# Autodesk Inventor assembly: Robot_assembly_full
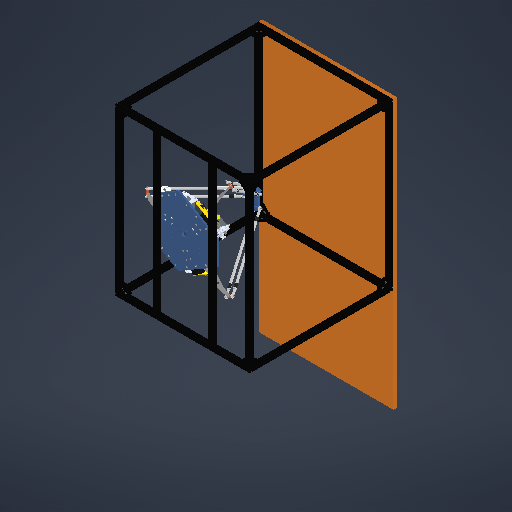
[picture p0: Inventor's stored thumbnail of the model, 512x512]
Saved by Autodesk Inventor 2027.1 (Build 311270010, 270A)
## iProperties
Created: 2026-08-09
Part Number: Robot_assembly_full
Document SubType Name: Assembly
Designer: MSI
Author: MSI
## Documents named in this file (35)
- C:\Users\MSI\Documents\MECHATRONICS\Tot_nghiep\Do_an_Delta.Robot_Dang_Rui_Bi\Thiết kế\Delta Part\Robot_assembly_full.iam
- C:\Users\MSI\Documents\MECHATRONICS\Tot_nghiep\Do_an_Delta.Robot_Dang_Rui_Bi\Thiết kế\Delta Part\tấm gỗ.ipt
- C:\Users\MSI\Documents\MECHATRONICS\Tot_nghiep\Do_an_Delta.Robot_Dang_Rui_Bi\Thiết kế\Delta Part\nhôm định hình 20x20_600.ipt
- C:\Users\MSI\Documents\MECHATRONICS\Tot_nghiep\Do_an_Delta.Robot_Dang_Rui_Bi\Thiết kế\Delta Part\nhôm định hình 20x20_700.ipt
- C:\Users\MSI\Documents\MECHATRONICS\Tot_nghiep\Do_an_Delta.Robot_Dang_Rui_Bi\Thiết kế\Delta Part\ke góc.ipt
- C:\Users\MSI\Documents\Inventor\Content Center Files\R2027\en-US\ISO 7380-1\ISO 7380-1 - M5 x 8.ipt
- C:\Users\MSI\Documents\MECHATRONICS\Tot_nghiep\Do_an_Delta.Robot_Dang_Rui_Bi\Thiết kế\Delta Part\nhôm định hình 20x20_600_có lỗ.ipt
- C:\Users\MSI\Documents\MECHATRONICS\Tot_nghiep\Do_an_Delta.Robot_Dang_Rui_Bi\Thiết kế\Delta Part\nhôm định hình 20x20_700_co lỗ1.ipt
- C:\Users\MSI\Documents\MECHATRONICS\Tot_nghiep\Do_an_Delta.Robot_Dang_Rui_Bi\Thiết kế\Delta Part\nhôm định hình 20x20_700_co lỗ2.ipt
- C:\Users\MSI\Documents\MECHATRONICS\Tot_nghiep\Do_an_Delta.Robot_Dang_Rui_Bi\Thiết kế\Delta Part\đế trên.ipt
- C:\Users\MSI\Documents\MECHATRONICS\Tot_nghiep\Do_an_Delta.Robot_Dang_Rui_Bi\Thiết kế\Delta Part\nhôm định hình đôi_gá link1.ipt
- C:\Users\MSI\Documents\MECHATRONICS\Tot_nghiep\Do_an_Delta.Robot_Dang_Rui_Bi\Thiết kế\Delta Part\Hộp trượt vòng bi.ipt
- C:\Users\MSI\Documents\MECHATRONICS\Tot_nghiep\Do_an_Delta.Robot_Dang_Rui_Bi\Thiết kế\Delta Part\trục đai.ipt
- C:\Users\MSI\Documents\MECHATRONICS\Tot_nghiep\Do_an_Delta.Robot_Dang_Rui_Bi\Thiết kế\Delta Part\mặt bích.ipt
- C:\Users\MSI\Documents\MECHATRONICS\Tot_nghiep\Do_an_Delta.Robot_Dang_Rui_Bi\Thiết kế\Delta Part\Link1.ipt
- C:\Users\MSI\Documents\MECHATRONICS\Tot_nghiep\Do_an_Delta.Robot_Dang_Rui_Bi\Thiết kế\Delta Part\khóa trục.ipt
- C:\Users\MSI\Documents\MECHATRONICS\Tot_nghiep\Do_an_Delta.Robot_Dang_Rui_Bi\Thiết kế\Delta Part\chốt khớp nối.ipt
- C:\Users\MSI\Documents\MECHATRONICS\Tot_nghiep\Do_an_Delta.Robot_Dang_Rui_Bi\Thiết kế\Delta Part\Base_E_buffer.ipt
- C:\Users\MSI\Documents\MECHATRONICS\Tot_nghiep\Do_an_Delta.Robot_Dang_Rui_Bi\Thiết kế\Delta Part\linh2_mawts traau.iam
- C:\Users\MSI\Documents\MECHATRONICS\Tot_nghiep\Do_an_Delta.Robot_Dang_Rui_Bi\Thiết kế\Delta Part\đế gá step.ipt
- C:\Users\MSI\Documents\MECHATRONICS\Tot_nghiep\Do_an_Delta.Robot_Dang_Rui_Bi\Thiết kế\Delta Part\nema23_57HS56\nema23.iam
- C:\Users\MSI\Documents\MECHATRONICS\Tot_nghiep\Do_an_Delta.Robot_Dang_Rui_Bi\Thiết kế\Delta Part\GT2_20T.ipt
- C:\Users\MSI\Documents\MECHATRONICS\Tot_nghiep\Do_an_Delta.Robot_Dang_Rui_Bi\Thiết kế\Delta Part\GT2_60.ipt
- C:\Users\MSI\Documents\Inventor\Content Center Files\R2027\en-US\AS 1427(05)\AS 1427 - M4 x 8(5) II.ipt
- C:\Users\MSI\Documents\Inventor\Content Center Files\R2027\en-US\AS 1427(05)\AS 1427 - M2.5 x 4(5) II.ipt
- C:\Users\MSI\Documents\Inventor\Content Center Files\R2027\en-US\AS 1427(05)\AS 1427 - M3.5 x 5(5) II.ipt
- C:\Users\MSI\Documents\Inventor\Content Center Files\R2027\en-US\AS 1427(05)\AS 1427 - M3 x 5(5) II.ipt
- C:\Users\MSI\Documents\Inventor\Content Center Files\R2027\en-US\AS 1427(05)\AS 1427 - M3 x 16(5) II.ipt
- C:\Users\MSI\Documents\Inventor\Content Center Files\R2027\en-US\AS 1427(05)\AS 1427 - M4 x 6(5) II.ipt
- C:\Users\MSI\Documents\Inventor\Content Center Files\R2027\en-US\ANSI B18.3.4M(1)\ANSI B18.3.4M - M3 x 0.5 x 45(2).ipt
- C:\Users\MSI\Documents\Inventor\Content Center Files\R2027\en-US\ANSI B18.2.4.2M\ANSI B18.2.4.2M - M3.5x0.6 - 6.ipt
- C:\Users\MSI\Documents\MECHATRONICS\Tot_nghiep\Do_an_Delta.Robot_Dang_Rui_Bi\Thiết kế\Tool_STL\Part1.ipt
- C:\Users\MSI\Documents\Inventor\Content Center Files\R2027\en-US\AS 1427(05)\AS 1427 - M4 x 10(5) II.ipt
- C:\Users\MSI\Documents\MECHATRONICS\Tot_nghiep\Do_an_Delta.Robot_Dang_Rui_Bi\Thiết kế\Delta Part\công tắc hành trình.ipt
- C:\Users\MSI\Documents\Inventor\Content Center Files\R2027\en-US\AS 1427(05)\AS 1427 - M4 x 16(5) II.ipt
## Components (233 placed, 34 different names)
1. tấm gỗ:1 — Flush:1, Mate:1, Flush:2, Mate:3, Flush:4, Mate:5, Flush:5, Flush:46, Flush:47, Flush:48
2. nhôm định hình 20x20_600:1 — Flush:1, Mate:1, Mate:2, Flush:3, Mate:4, Mate:10, Flush:10, Flush:11, Mate:11, Flush:12, Flush:13, Mate:21, Mate:22, Flush:24, Mate:27, Mate:30, Flush:28, Flush:47
3. nhôm định hình 20x20_700:1 — Mate:2, Flush:2, Flush:3, Mate:7, Mate:19, Mate:20, Flush:22, Flush:23, Mate:32, Flush:29, Mate:36, Flush:46
4. nhôm định hình 20x20_700:2 — Mate:3, Flush:4, Mate:4, Mate:6, Mate:8, Flush:6, Mate:23, Mate:25, Mate:28, Mate:38, Flush:48
5. nhôm định hình 20x20_600:2 — Mate:5, Mate:6, Mate:7, Flush:5, Flush:7, Mate:9, Flush:8, Flush:9, Mate:18, Mate:24, Flush:25, Mate:35, Mate:40
6. nhôm định hình 20x20_600:3 — Mate:10, Flush:10, Flush:11, Mate:31, Mate:33, Mate:54, Mate:56, Flush:41, Flush:50, Flush:53, Flush:54
7. nhôm định hình 20x20_600:4 — Mate:11, Flush:12, Flush:13, Mate:26, Flush:26, Mate:29, Flush:27, Mate:50, Mate:52, Flush:55, Flush:57, Flush:73
8. nhôm định hình 20x20_600:5 — Mate:9, Flush:8, Flush:9, Mate:34, Flush:30, Mate:37, Flush:31, Mate:43, Flush:34, Mate:44, Mate:67, Flush:59
9. nhôm định hình 20x20_600:6 — Mate:8, Flush:6, Flush:7, Mate:39, Flush:32, Mate:41, Flush:33, Mate:46, Flush:36, Mate:48, Flush:58
10. nhôm định hình 20x20_700:3 — Mate:45, Flush:35, Mate:57, Mate:58, Mate:60, Flush:49, Flush:60, Flush:67, Mate:73
11. nhôm định hình 20x20_700:4 — Mate:49, Flush:37, Mate:51, Flush:38, Mate:63, Flush:44, Mate:65, Mate:66, Flush:56, Flush:61, Flush:68, Flush:70
12. ke góc:1 — Mate:28, Mate:29, Flush:27, Insert:23, Insert:24
13. ke góc:2 — Mate:32, Mate:33, Flush:29, Insert:31, Insert:32
14. ke góc:3 — Mate:38, Mate:39, Flush:32, Insert:5, Insert:6, Insert:9
15. ke góc:4 — Mate:36, Mate:37, Flush:31, Insert:12, Insert:13
16. ke góc:5 — Mate:34, Mate:35, Flush:30, Insert:16, Insert:17
17. ke góc:6 — Mate:26, Mate:27, Flush:26, Insert:21, Insert:22
18. ke góc:7 — Mate:24, Mate:25, Flush:25, Insert:1, Insert:2, Insert:3, Insert:4
19. ke góc:8 — Mate:18, Mate:19, Flush:23, Insert:14, Insert:15
20. ke góc:9 — Mate:22, Flush:24, Mate:23, Insert:25, Insert:26
21. ke góc:10 — Mate:20, Mate:21, Flush:22, Insert:29, Insert:30
22. ke góc:11 — Mate:30, Mate:31, Flush:28, Insert:33, Insert:34
23. ke góc:12 — Mate:46, Flush:36, Insert:39, Insert:40, Flush:63, Mate:74
24. ke góc:13 — Mate:58, Insert:54, Insert:55, Flush:65, Mate:72
25. ke góc:14 — Mate:56, Mate:57, Flush:41, Insert:47, Insert:52
26. ke góc:15 — Mate:52, Insert:41, Insert:42, Flush:73, Mate:70
27. ke góc:16 — Mate:48, Mate:49, Flush:37, Insert:35, Insert:37
28. ke góc:17 — Mate:50, Mate:51, Flush:38, Insert:45, Insert:46
29. ke góc:18 — Mate:44, Mate:45, Flush:35, Insert:57, Insert:58
30. ke góc:19 — Mate:43, Flush:34, Insert:53, Insert:56, Flush:62, Mate:75
31. ke góc:20 — Mate:54, Insert:50, Insert:51, Mate:69, Flush:72
32. ke góc:21 — Mate:40, Mate:41, Flush:33, Insert:7, Insert:8
33. ke góc:22 — Mate:60, Insert:48, Insert:49, Flush:66, Flush:67, Mate:76
34. ke góc:23 — Mate:63, Flush:44, Insert:43, Insert:44, Mate:68, Flush:68, Flush:69
35. ke góc:24 — Mate:65, Insert:36, Insert:38, Flush:64, Flush:70, Flush:71, Mate:71
36. ISO 7380-1 M5 x 8:1 — Insert:1
37. ISO 7380-1 M5 x 8:2 — Insert:2
38. ISO 7380-1 M5 x 8:3 — Insert:3
39. ISO 7380-1 M5 x 8:4 — Insert:4
40. ISO 7380-1 M5 x 8:5 — Insert:5
41. ISO 7380-1 M5 x 8:6 — Insert:6
42. ISO 7380-1 M5 x 8:7 — Insert:7
43. ISO 7380-1 M5 x 8:8 — Insert:8
44. ISO 7380-1 M5 x 8:9 — Insert:9
45. ISO 7380-1 M5 x 8:12 — Insert:12
46. ISO 7380-1 M5 x 8:13 — Insert:13
47. ISO 7380-1 M5 x 8:14 — Insert:14
48. ISO 7380-1 M5 x 8:15 — Insert:15
49. ISO 7380-1 M5 x 8:16 — Insert:16
50. ISO 7380-1 M5 x 8:17 — Insert:17
51. ISO 7380-1 M5 x 8:22 — Insert:21
52. ISO 7380-1 M5 x 8:23 — Insert:22
53. ISO 7380-1 M5 x 8:24 — Insert:23
54. ISO 7380-1 M5 x 8:25 — Insert:24
55. ISO 7380-1 M5 x 8:26 — Insert:25
56. ISO 7380-1 M5 x 8:27 — Insert:26
57. ISO 7380-1 M5 x 8:30 — Insert:29
58. ISO 7380-1 M5 x 8:31 — Insert:30
59. ISO 7380-1 M5 x 8:32 — Insert:31
60. ISO 7380-1 M5 x 8:33 — Insert:32
61. ISO 7380-1 M5 x 8:34 — Insert:33
62. ISO 7380-1 M5 x 8:35 — Insert:34
63. ISO 7380-1 M5 x 8:36 — Insert:35
64. ISO 7380-1 M5 x 8:37 — Insert:36
65. ISO 7380-1 M5 x 8:38 — Insert:37
66. ISO 7380-1 M5 x 8:39 — Insert:38
67. ISO 7380-1 M5 x 8:40 — Insert:39
68. ISO 7380-1 M5 x 8:41 — Insert:40
69. ISO 7380-1 M5 x 8:42 — Insert:41
70. ISO 7380-1 M5 x 8:43 — Insert:42
71. ISO 7380-1 M5 x 8:44 — Insert:43
72. ISO 7380-1 M5 x 8:45 — Insert:44
73. ISO 7380-1 M5 x 8:46 — Insert:45
74. ISO 7380-1 M5 x 8:47 — Insert:46
75. ISO 7380-1 M5 x 8:48 — Insert:47
76. ISO 7380-1 M5 x 8:49 — Insert:48
77. ISO 7380-1 M5 x 8:50 — Insert:49
78. ISO 7380-1 M5 x 8:51 — Insert:50
79. ISO 7380-1 M5 x 8:52 — Insert:51
80. ISO 7380-1 M5 x 8:53 — Insert:52
81. ISO 7380-1 M5 x 8:54 — Insert:53
82. ISO 7380-1 M5 x 8:55 — Insert:54
83. ISO 7380-1 M5 x 8:56 — Insert:55
84. ISO 7380-1 M5 x 8:57 — Insert:56
85. ISO 7380-1 M5 x 8:58 — Insert:57
86. ISO 7380-1 M5 x 8:59 — Insert:58
87. nhôm định hình 20x20_600_có lỗ:1 — Mate:66, Mate:67, Flush:49, Flush:58, Flush:59, Flush:60, Flush:61, Flush:62, Flush:63, Flush:64, Flush:65, Flush:71, Mate:71, Mate:72, Mate:73, Mate:74, Mate:75, Mate:78, Flush:74, Mate:79
88. nhôm định hình 20x20_600_có lỗ:2 — Mate:68, Mate:69, Flush:50, Flush:53, Flush:54, Flush:55, Flush:56, Flush:57, Flush:66, Flush:69, Flush:72, Mate:70, Mate:76, Mate:77, Flush:75, Mate:80
89. nhôm định hình 20x20_700_co lỗ1:1 — Mate:77, Mate:78, Flush:74, Mate:81
90. nhôm định hình 20x20_700_co lỗ2:1 — Mate:79, Flush:75, Mate:80, Flush:76, Mate:82, Insert:104, Insert:105, Insert:106
91. đế trên:1 — Mate:81, Flush:76, Mate:82, Mate:83, Mate:84, Mate:85, Mate:95, Mate:96, Mate:97, Mate:98, Mate:99, Mate:100, Insert:94, Insert:95, Insert:96, Insert:97, Insert:98, Insert:99, Insert:100, Insert:101, Insert:103, Insert:107, Insert:108, Insert:109, Insert:110, Insert:111, Insert:141, Insert:142, Insert:143, Insert:144, Insert:145, Insert:146, Insert:147, Insert:148, Insert:149, Insert:150, Insert:151, Insert:152, Insert:153
92. nhôm định hình đôi_gá link1:1 — Mate:83, Mate:84, Mate:85, Mate:86, Flush:77, Flush:82, Mate:236, Flush:83, Flush:84, Flush:103, Flush:104, Mate:265
93. Hộp trượt vòng bi:1 — Mate:86, Flush:77, Mate:88, Mate:89, Mate:122, Flush:82, Insert:90, Insert:91, Insert:92, Insert:93
94. trục đai:1 — Mate:88, Mate:89, Mate:90, Mate:121, Mate:209, Mate:256
95. mặt bích:1 — Mate:90, Mate:92, Mate:93, Mate:94, Mate:209
96. Link1:1 — Mate:92, Mate:93, Mate:94, Mate:129, Mate:130, Mate:131, Mate:132, Insert:79, Insert:80, Insert:81, Insert:82
97. nhôm định hình đôi_gá link1:2 — Mate:98, Mate:99, Mate:100, Mate:101, Flush:78, Flush:80, Flush:87, Mate:242, Flush:88, Mate:266, Flush:105, Flush:106
98. nhôm định hình đôi_gá link1:3 — Mate:95, Mate:96, Mate:97, Mate:103, Flush:79, Flush:81, Mate:239, Flush:86, Flush:94, Mate:267, Flush:107, Flush:108
99. Hộp trượt vòng bi:2 — Mate:101, Flush:78, Mate:107, Mate:124, Flush:80, Insert:83, Insert:84, Insert:85, Insert:86
100. Hộp trượt vòng bi:3 — Mate:103, Flush:79, Mate:105, Mate:106, Mate:120, Flush:81, Mate:261, Mate:262, Insert:87, Insert:88, Insert:89
101. trục đai:2 — Mate:105, Mate:106, Mate:111, Mate:119, Mate:208, Mate:257
102. trục đai:3 — Mate:107, Mate:109, Mate:123, Mate:255
103. mặt bích:2 — Mate:111, Mate:116, Mate:117, Mate:118, Mate:208
104. mặt bích:3 — Mate:109, Mate:113, Mate:114, Mate:115
105. Link1:2 — Mate:113, Mate:114, Mate:115, Mate:133, Mate:134, Mate:135, Mate:136, Insert:75, Insert:76, Insert:77, Insert:78
106. Link1:3 — Mate:116, Mate:117, Mate:118, Mate:125, Mate:126, Mate:127, Mate:128, Insert:71, Insert:72, Insert:73, Insert:74
107. khóa trục:1 — Mate:119, Mate:120, Mate:258
108. khóa trục:2 — Mate:121, Mate:122, Mate:259
109. khóa trục:3 — Mate:123, Mate:124, Mate:260
110. chốt khớp nối:1 — Mate:125, Mate:126, Mate:215
111. chốt khớp nối:2 — Mate:131, Mate:132, Mate:212, Mate:213
112. chốt khớp nối:3 — Mate:127, Mate:128, Mate:214, Mate:216, Mate:217
113. chốt khớp nối:4 — Mate:135, Mate:136, Mate:218, Mate:219
114. chốt khớp nối:5 — Mate:133, Mate:134, Mate:220, Mate:221
115. chốt khớp nối:6 — Mate:129, Mate:130, Mate:210, Mate:211
116. linh2_mawts traau:1 [sub-assembly] — Mate:210, Mate:211, Mate:232, Mate:233, Insert:131, Insert:132
117. linh2_mawts traau:2 [sub-assembly] — Mate:218, Mate:219, Mate:227, Mate:228, Insert:129, Insert:133
118. linh2_mawts traau:3 [sub-assembly] — Mate:216, Mate:217, Mate:224, Mate:231, Insert:126, Mate:263, Mate:264
119. linh2_mawts traau:4 [sub-assembly] — Mate:220, Mate:221, Mate:225, Mate:226, Mate:229, Insert:127, Insert:128
120. linh2_mawts traau:5 [sub-assembly] — Mate:214, Mate:215, Mate:222, Mate:223, Mate:230, Insert:130, Insert:134
121. linh2_mawts traau:6 [sub-assembly] — Mate:212, Mate:213, Mate:234, Mate:235, Insert:124, Insert:125
122. Base_E_buffer:1 — Mate:222, Mate:223, Mate:224, Mate:225, Mate:226, Mate:227, Mate:228, Mate:229, Mate:230, Mate:231, Mate:232, Mate:233, Mate:234, Mate:235
123. nema23:1 [sub-assembly] — Mate:237, Mate:251, Mate:252, Flush:97
124. đế gá step:1 — Mate:236, Flush:83, Flush:84, Mate:237, Mate:251, Insert:63, Insert:64, Insert:65, Insert:66
125. đế gá step:2 — Mate:239, Flush:86, Flush:94, Mate:249, Flush:96, Insert:59, Insert:60, Insert:61, Insert:62
126. đế gá step:3 — Flush:87, Mate:242, Flush:88, Mate:243, Flush:95, Insert:67, Insert:68, Insert:69, Insert:70
127. nema23:3 [sub-assembly] — Mate:243, Flush:95, Mate:254, Flush:99
128. nema23:4 [sub-assembly] — Mate:249, Flush:96, Mate:253, Flush:98
129. GT2_20T:1 — Mate:253, Flush:98, Flush:102
130. GT2_20T:2 — Mate:252, Flush:97, Flush:101
131. GT2_20T:3 — Mate:254, Flush:99, Flush:100
132. GT2_60:1 — Mate:257, Flush:102
133. GT2_60:2 — Mate:255, Flush:100
134. GT2_60:3 — Mate:256, Flush:101
135. AS 1427 H - Metric M4 x 8:1 — Insert:59
136. AS 1427 H - Metric M4 x 8:2 — Insert:60
137. AS 1427 H - Metric M4 x 8:3 — Insert:61
138. AS 1427 H - Metric M4 x 8:4 — Insert:62
139. AS 1427 H - Metric M4 x 8:5 — Insert:63
140. AS 1427 H - Metric M4 x 8:6 — Insert:64
141. AS 1427 H - Metric M4 x 8:7 — Insert:65
142. AS 1427 H - Metric M4 x 8:8 — Insert:66
143. AS 1427 H - Metric M4 x 8:9 — Insert:67
144. AS 1427 H - Metric M4 x 8:10 — Insert:68
145. AS 1427 H - Metric M4 x 8:11 — Insert:69
146. AS 1427 H - Metric M4 x 8:12 — Insert:70
147. AS 1427 H - Metric M2.5 x 4:1 — Insert:71
148. AS 1427 H - Metric M2.5 x 4:2 — Insert:72
149. AS 1427 H - Metric M2.5 x 4:3 — Insert:73
150. AS 1427 H - Metric M2.5 x 4:4 — Insert:74
151. AS 1427 H - Metric M2.5 x 4:5 — Insert:75
152. AS 1427 H - Metric M2.5 x 4:6 — Insert:76
153. AS 1427 H - Metric M2.5 x 4:7 — Insert:77
154. AS 1427 H - Metric M2.5 x 4:8 — Insert:78
155. AS 1427 H - Metric M2.5 x 4:9 — Insert:79
156. AS 1427 H - Metric M2.5 x 4:10 — Insert:80
157. AS 1427 H - Metric M2.5 x 4:11 — Insert:81
158. AS 1427 H - Metric M2.5 x 4:12 — Insert:82
159. AS 1427 H - Metric M3.5 x 5:1 — Mate:258
160. AS 1427 H - Metric M3.5 x 5:2 — Mate:259
161. AS 1427 H - Metric M3.5 x 5:3 — Mate:260
162. AS 1427 H - Metric M3 x 5:1 — Insert:83
163. AS 1427 H - Metric M3 x 5:2 — Insert:84
164. AS 1427 H - Metric M3 x 5:3 — Insert:85
165. AS 1427 H - Metric M3 x 5:4 — Insert:86
166. AS 1427 H - Metric M3 x 5:5 — Mate:261, Mate:262
167. AS 1427 H - Metric M3 x 5:6 — Insert:87
168. AS 1427 H - Metric M3 x 5:7 — Insert:88
169. AS 1427 H - Metric M3 x 16:1 — Insert:89
170. AS 1427 H - Metric M3 x 16:2 — Insert:90
171. AS 1427 H - Metric M3 x 16:3 — Insert:91
172. AS 1427 H - Metric M3 x 16:4 — Insert:92
173. AS 1427 H - Metric M3 x 16:5 — Insert:93
174. AS 1427 H - Metric M4 x 6:1 — Insert:94
175. AS 1427 H - Metric M4 x 6:2 — Insert:95
176. AS 1427 H - Metric M4 x 6:3 — Insert:96
177. AS 1427 H - Metric M4 x 6:4 — Insert:97
178. AS 1427 H - Metric M4 x 6:5 — Insert:98
179. AS 1427 H - Metric M4 x 6:6 — Insert:99
180. AS 1427 H - Metric M4 x 6:7 — Insert:100
181. AS 1427 H - Metric M4 x 6:8 — Insert:101
182. AS 1427 H - Metric M4 x 6:10 — Insert:103
183. AS 1427 H - Metric M4 x 6:11 — Insert:104
184. AS 1427 H - Metric M4 x 6:12 — Insert:105
185. AS 1427 H - Metric M4 x 6:13 — Insert:106
186. AS 1427 H - Metric M4 x 6:14 — Insert:107
187. AS 1427 H - Metric M4 x 6:15 — Insert:108
188. AS 1427 H - Metric M4 x 6:16 — Insert:109
189. AS 1427 H - Metric M4 x 6:17 — Insert:110
190. AS 1427 H - Metric M4 x 6:18 — Insert:111
191. Broached Hexagon Socket Button Head Cap Screw - Metric M3 x 0.5 x 45:1 — Insert:124
192. Broached Hexagon Socket Button Head Cap Screw - Metric M3 x 0.5 x 45:2 — Insert:125
193. Broached Hexagon Socket Button Head Cap Screw - Metric M3 x 0.5 x 45:3 — Insert:126
194. Broached Hexagon Socket Button Head Cap Screw - Metric M3 x 0.5 x 45:4 — Mate:263, Mate:264
195. Broached Hexagon Socket Button Head Cap Screw - Metric M3 x 0.5 x 45:5 — Insert:127
196. Broached Hexagon Socket Button Head Cap Screw - Metric M3 x 0.5 x 45:6 — Insert:128
197. ANSI B18.2.4.2M M3.5x0.6:1 — Insert:129
198. ANSI B18.2.4.2M M3.5x0.6:2 — Insert:130
199. ANSI B18.2.4.2M M3.5x0.6:3 — Insert:131
200. ANSI B18.2.4.2M M3.5x0.6:4 — Insert:132
201. ANSI B18.2.4.2M M3.5x0.6:5 — Insert:133
202. ANSI B18.2.4.2M M3.5x0.6:6 — Insert:134
203. Part1:1 — Mate:266, Flush:105, Flush:106, Insert:139, Insert:140, Mate:274, Mate:275, Mate:276
204. Part1:2 — Mate:267, Flush:107, Flush:108, Insert:135, Insert:136, Mate:271, Mate:272, Mate:273
205. Part1:3 — Flush:103, Flush:104, Mate:265, Insert:137, Insert:138, Mate:268, Mate:269, Mate:270
206. AS 1427 H - Metric M4 x 10:1 — Insert:135
207. AS 1427 H - Metric M4 x 10:2 — Insert:136
208. AS 1427 H - Metric M4 x 10:3 — Insert:137
209. AS 1427 H - Metric M4 x 10:4 — Insert:138
210. AS 1427 H - Metric M4 x 10:5 — Insert:139
211. AS 1427 H - Metric M4 x 10:6 — Insert:140
212. công tắc hành trình:1 — Mate:271, Mate:272, Mate:273, Insert:154, Insert:155
213. công tắc hành trình:2 — Mate:274, Mate:275, Mate:276, Insert:156, Insert:157
214. công tắc hành trình:3 — Mate:268, Mate:269, Mate:270, Insert:158, Insert:159
215. AS 1427 H - Metric M4 x 16:1 — Insert:141
216. AS 1427 H - Metric M4 x 16:2 — Insert:142
217. AS 1427 H - Metric M4 x 16:3 — Insert:143
218. AS 1427 H - Metric M4 x 16:4 — Insert:144
219. AS 1427 H - Metric M4 x 16:5 — Insert:145
220. AS 1427 H - Metric M4 x 16:6 — Insert:146
221. AS 1427 H - Metric M4 x 16:7 — Insert:147
222. AS 1427 H - Metric M4 x 16:8 — Insert:148
223. AS 1427 H - Metric M4 x 16:9 — Insert:149
224. AS 1427 H - Metric M4 x 16:10 — Insert:150
225. AS 1427 H - Metric M4 x 16:11 — Insert:151
226. AS 1427 H - Metric M4 x 10:7 — Insert:152
227. AS 1427 H - Metric M4 x 16:12 — Insert:153
228. AS 1427 H - Metric M3 x 5:8 — Insert:154
229. AS 1427 H - Metric M3 x 5:9 — Insert:155
230. AS 1427 H - Metric M3 x 5:10 — Insert:156
231. AS 1427 H - Metric M3 x 5:11 — Insert:157
232. AS 1427 H - Metric M3 x 5:12 — Insert:158
233. AS 1427 H - Metric M3 x 5:13 — Insert:159
## Relationships (401: Mate 175, Insert 139, Flush 87)
- Flush:1: tấm gỗ:1 ↔ nhôm định hình 20x20_600:1
- Mate:1: tấm gỗ:1 ↔ nhôm định hình 20x20_600:1
- Mate:2: nhôm định hình 20x20_600:1 ↔ nhôm định hình 20x20_700:1
- Flush:2: tấm gỗ:1 ↔ nhôm định hình 20x20_700:1
- Flush:3: nhôm định hình 20x20_600:1 ↔ nhôm định hình 20x20_700:1
- Mate:3: tấm gỗ:1 ↔ nhôm định hình 20x20_700:2
- Flush:4: tấm gỗ:1 ↔ nhôm định hình 20x20_700:2
- Mate:4: nhôm định hình 20x20_600:1 ↔ nhôm định hình 20x20_700:2
- Mate:5: tấm gỗ:1 ↔ nhôm định hình 20x20_600:2
- Mate:6: nhôm định hình 20x20_700:2 ↔ nhôm định hình 20x20_600:2
- Mate:7: nhôm định hình 20x20_700:1 ↔ nhôm định hình 20x20_600:2
- Flush:5: tấm gỗ:1 ↔ nhôm định hình 20x20_600:2
- Mate:8: nhôm định hình 20x20_700:2 ↔ nhôm định hình 20x20_600:6
- Flush:6: nhôm định hình 20x20_700:2 ↔ nhôm định hình 20x20_600:6
- Flush:7: nhôm định hình 20x20_600:2 ↔ nhôm định hình 20x20_600:6
- Mate:9: nhôm định hình 20x20_600:2 ↔ nhôm định hình 20x20_600:5
- Flush:8: nhôm định hình 20x20_600:2 ↔ nhôm định hình 20x20_600:5
- Flush:9: nhôm định hình 20x20_600:2 ↔ nhôm định hình 20x20_600:5
- Mate:10: nhôm định hình 20x20_600:1 ↔ nhôm định hình 20x20_600:3
- Flush:10: nhôm định hình 20x20_600:1 ↔ nhôm định hình 20x20_600:3
- Flush:11: nhôm định hình 20x20_600:1 ↔ nhôm định hình 20x20_600:3
- Mate:11: nhôm định hình 20x20_600:1 ↔ nhôm định hình 20x20_600:4
- Flush:12: nhôm định hình 20x20_600:1 ↔ nhôm định hình 20x20_600:4
- Flush:13: nhôm định hình 20x20_600:1 ↔ nhôm định hình 20x20_600:4
- Mate:18: nhôm định hình 20x20_600:2 ↔ ke góc:8
- Mate:19: nhôm định hình 20x20_700:1 ↔ ke góc:8
- Mate:20: nhôm định hình 20x20_700:1 ↔ ke góc:10
- Mate:21: nhôm định hình 20x20_600:1 ↔ ke góc:10
- Flush:22: nhôm định hình 20x20_700:1 ↔ ke góc:10
- Flush:23: nhôm định hình 20x20_700:1 ↔ ke góc:8
- Mate:22: nhôm định hình 20x20_600:1 ↔ ke góc:9
- Flush:24: nhôm định hình 20x20_600:1 ↔ ke góc:9
- Mate:23: nhôm định hình 20x20_700:2 ↔ ke góc:9
- Mate:24: nhôm định hình 20x20_600:2 ↔ ke góc:7
- Mate:25: nhôm định hình 20x20_700:2 ↔ ke góc:7
- Flush:25: nhôm định hình 20x20_600:2 ↔ ke góc:7
- Mate:26: nhôm định hình 20x20_600:4 ↔ ke góc:6
- Mate:27: nhôm định hình 20x20_600:1 ↔ ke góc:6
- Flush:26: nhôm định hình 20x20_600:4 ↔ ke góc:6
- Mate:28: nhôm định hình 20x20_700:2 ↔ ke góc:1
- Mate:29: nhôm định hình 20x20_600:4 ↔ ke góc:1
- Flush:27: nhôm định hình 20x20_600:4 ↔ ke góc:1
- Mate:30: nhôm định hình 20x20_600:1 ↔ ke góc:11
- Mate:31: nhôm định hình 20x20_600:3 ↔ ke góc:11
- Flush:28: nhôm định hình 20x20_600:1 ↔ ke góc:11
- Mate:32: nhôm định hình 20x20_700:1 ↔ ke góc:2
- Mate:33: nhôm định hình 20x20_600:3 ↔ ke góc:2
- Flush:29: nhôm định hình 20x20_700:1 ↔ ke góc:2
- Mate:34: nhôm định hình 20x20_600:5 ↔ ke góc:5
- Mate:35: nhôm định hình 20x20_600:2 ↔ ke góc:5
- Flush:30: nhôm định hình 20x20_600:5 ↔ ke góc:5
- Mate:36: nhôm định hình 20x20_700:1 ↔ ke góc:4
- Mate:37: nhôm định hình 20x20_600:5 ↔ ke góc:4
- Flush:31: nhôm định hình 20x20_600:5 ↔ ke góc:4
- Mate:38: nhôm định hình 20x20_700:2 ↔ ke góc:3
- Mate:39: nhôm định hình 20x20_600:6 ↔ ke góc:3
- Flush:32: nhôm định hình 20x20_600:6 ↔ ke góc:3
- Mate:40: nhôm định hình 20x20_600:2 ↔ ke góc:21
- Mate:41: nhôm định hình 20x20_600:6 ↔ ke góc:21
- Flush:33: nhôm định hình 20x20_600:6 ↔ ke góc:21
- Mate:43: nhôm định hình 20x20_600:5 ↔ ke góc:19
- Flush:34: nhôm định hình 20x20_600:5 ↔ ke góc:19
- Mate:44: nhôm định hình 20x20_600:5 ↔ ke góc:18
- Mate:45: nhôm định hình 20x20_700:3 ↔ ke góc:18
- Flush:35: nhôm định hình 20x20_700:3 ↔ ke góc:18
- Mate:46: nhôm định hình 20x20_600:6 ↔ ke góc:12
- Flush:36: nhôm định hình 20x20_600:6 ↔ ke góc:12
- Mate:48: nhôm định hình 20x20_600:6 ↔ ke góc:16
- Mate:49: nhôm định hình 20x20_700:4 ↔ ke góc:16
- Flush:37: nhôm định hình 20x20_700:4 ↔ ke góc:16
- Mate:50: nhôm định hình 20x20_600:4 ↔ ke góc:17
- Mate:51: nhôm định hình 20x20_700:4 ↔ ke góc:17
- Flush:38: nhôm định hình 20x20_700:4 ↔ ke góc:17
- Mate:52: nhôm định hình 20x20_600:4 ↔ ke góc:15
- Mate:54: nhôm định hình 20x20_600:3 ↔ ke góc:20
- Mate:56: nhôm định hình 20x20_600:3 ↔ ke góc:14
- Mate:57: nhôm định hình 20x20_700:3 ↔ ke góc:14
- Flush:41: nhôm định hình 20x20_600:3 ↔ ke góc:14
- Mate:58: nhôm định hình 20x20_700:3 ↔ ke góc:13
- Mate:60: nhôm định hình 20x20_700:3 ↔ ke góc:22
- Mate:63: nhôm định hình 20x20_700:4 ↔ ke góc:23
- Flush:44: nhôm định hình 20x20_700:4 ↔ ke góc:23
- Mate:65: nhôm định hình 20x20_700:4 ↔ ke góc:24
- Insert:1: ke góc:7 ↔ ISO 7380-1 M5 x 8:1
- Insert:2: ke góc:7 ↔ ISO 7380-1 M5 x 8:2
- Insert:3: ke góc:7 ↔ ISO 7380-1 M5 x 8:3
- Insert:4: ke góc:7 ↔ ISO 7380-1 M5 x 8:4
- Insert:5: ke góc:3 ↔ ISO 7380-1 M5 x 8:5
- Insert:6: ke góc:3 ↔ ISO 7380-1 M5 x 8:6
- Insert:7: ke góc:21 ↔ ISO 7380-1 M5 x 8:7
- Insert:8: ke góc:21 ↔ ISO 7380-1 M5 x 8:8
- Insert:9: ke góc:3 ↔ ISO 7380-1 M5 x 8:9
- Insert:12: ke góc:4 ↔ ISO 7380-1 M5 x 8:12
- Insert:13: ke góc:4 ↔ ISO 7380-1 M5 x 8:13
- Insert:14: ke góc:8 ↔ ISO 7380-1 M5 x 8:14
- Insert:15: ke góc:8 ↔ ISO 7380-1 M5 x 8:15
- Insert:16: ke góc:5 ↔ ISO 7380-1 M5 x 8:16
- Insert:17: ke góc:5 ↔ ISO 7380-1 M5 x 8:17
- Insert:21: ke góc:6 ↔ ISO 7380-1 M5 x 8:22
- Insert:22: ke góc:6 ↔ ISO 7380-1 M5 x 8:23
- Insert:23: ke góc:1 ↔ ISO 7380-1 M5 x 8:24
- Insert:24: ke góc:1 ↔ ISO 7380-1 M5 x 8:25
- Insert:25: ke góc:9 ↔ ISO 7380-1 M5 x 8:26
- Insert:26: ke góc:9 ↔ ISO 7380-1 M5 x 8:27
- Insert:29: ke góc:10 ↔ ISO 7380-1 M5 x 8:30
- Insert:30: ke góc:10 ↔ ISO 7380-1 M5 x 8:31
- Insert:31: ke góc:2 ↔ ISO 7380-1 M5 x 8:32
- Insert:32: ke góc:2 ↔ ISO 7380-1 M5 x 8:33
- Insert:33: ke góc:11 ↔ ISO 7380-1 M5 x 8:34
- Insert:34: ke góc:11 ↔ ISO 7380-1 M5 x 8:35
- Insert:35: ke góc:16 ↔ ISO 7380-1 M5 x 8:36
- Insert:36: ke góc:24 ↔ ISO 7380-1 M5 x 8:37
- Insert:37: ke góc:16 ↔ ISO 7380-1 M5 x 8:38
- Insert:38: ke góc:24 ↔ ISO 7380-1 M5 x 8:39
- Insert:39: ke góc:12 ↔ ISO 7380-1 M5 x 8:40
- Insert:40: ke góc:12 ↔ ISO 7380-1 M5 x 8:41
- Insert:41: ke góc:15 ↔ ISO 7380-1 M5 x 8:42
- Insert:42: ke góc:15 ↔ ISO 7380-1 M5 x 8:43
- Insert:43: ke góc:23 ↔ ISO 7380-1 M5 x 8:44
- Insert:44: ke góc:23 ↔ ISO 7380-1 M5 x 8:45
- Insert:45: ke góc:17 ↔ ISO 7380-1 M5 x 8:46
- Insert:46: ke góc:17 ↔ ISO 7380-1 M5 x 8:47
- Insert:47: ke góc:14 ↔ ISO 7380-1 M5 x 8:48
- Insert:48: ke góc:22 ↔ ISO 7380-1 M5 x 8:49
- Insert:49: ke góc:22 ↔ ISO 7380-1 M5 x 8:50
- Insert:50: ke góc:20 ↔ ISO 7380-1 M5 x 8:51
- Insert:51: ke góc:20 ↔ ISO 7380-1 M5 x 8:52
- Insert:52: ke góc:14 ↔ ISO 7380-1 M5 x 8:53
- Insert:53: ke góc:19 ↔ ISO 7380-1 M5 x 8:54
- Insert:54: ke góc:13 ↔ ISO 7380-1 M5 x 8:55
- Insert:55: ke góc:13 ↔ ISO 7380-1 M5 x 8:56
- Insert:56: ke góc:19 ↔ ISO 7380-1 M5 x 8:57
- Insert:57: ke góc:18 ↔ ISO 7380-1 M5 x 8:58
- Insert:58: ke góc:18 ↔ ISO 7380-1 M5 x 8:59
- Flush:46: tấm gỗ:1 ↔ nhôm định hình 20x20_700:1
- Flush:47: tấm gỗ:1 ↔ nhôm định hình 20x20_600:1
- Flush:48: tấm gỗ:1 ↔ nhôm định hình 20x20_700:2
- Mate:66: nhôm định hình 20x20_700:4 ↔ nhôm định hình 20x20_600_có lỗ:1
- Mate:67: nhôm định hình 20x20_600:5 ↔ nhôm định hình 20x20_600_có lỗ:1
- Flush:49: nhôm định hình 20x20_700:3 ↔ nhôm định hình 20x20_600_có lỗ:1
- Mate:68: ke góc:23 ↔ nhôm định hình 20x20_600_có lỗ:2
- Mate:69: ke góc:20 ↔ nhôm định hình 20x20_600_có lỗ:2
- Flush:50: nhôm định hình 20x20_600:3 ↔ nhôm định hình 20x20_600_có lỗ:2
- Flush:53: nhôm định hình 20x20_600:3 ↔ nhôm định hình 20x20_600_có lỗ:2
- Flush:54: nhôm định hình 20x20_600:3 ↔ nhôm định hình 20x20_600_có lỗ:2
- Flush:55: nhôm định hình 20x20_600:4 ↔ nhôm định hình 20x20_600_có lỗ:2
- Flush:56: nhôm định hình 20x20_700:4 ↔ nhôm định hình 20x20_600_có lỗ:2
- Flush:57: nhôm định hình 20x20_600:4 ↔ nhôm định hình 20x20_600_có lỗ:2
- Flush:58: nhôm định hình 20x20_600:6 ↔ nhôm định hình 20x20_600_có lỗ:1
- Flush:59: nhôm định hình 20x20_600:5 ↔ nhôm định hình 20x20_600_có lỗ:1
- Flush:60: nhôm định hình 20x20_700:3 ↔ nhôm định hình 20x20_600_có lỗ:1
- Flush:61: nhôm định hình 20x20_700:4 ↔ nhôm định hình 20x20_600_có lỗ:1
- Flush:62: ke góc:19 ↔ nhôm định hình 20x20_600_có lỗ:1
- Flush:63: ke góc:12 ↔ nhôm định hình 20x20_600_có lỗ:1
- Flush:64: ke góc:24 ↔ nhôm định hình 20x20_600_có lỗ:1
- Flush:65: ke góc:13 ↔ nhôm định hình 20x20_600_có lỗ:1
- Flush:66: ke góc:22 ↔ nhôm định hình 20x20_600_có lỗ:2
- Flush:67: nhôm định hình 20x20_700:3 ↔ ke góc:22
- Flush:68: nhôm định hình 20x20_700:4 ↔ ke góc:23
- Flush:69: ke góc:23 ↔ nhôm định hình 20x20_600_có lỗ:2
- Flush:70: nhôm định hình 20x20_700:4 ↔ ke góc:24
- Flush:71: ke góc:24 ↔ nhôm định hình 20x20_600_có lỗ:1
- Flush:72: ke góc:20 ↔ nhôm định hình 20x20_600_có lỗ:2
- Flush:73: nhôm định hình 20x20_600:4 ↔ ke góc:15
- Mate:70: ke góc:15 ↔ nhôm định hình 20x20_600_có lỗ:2
- Mate:71: ke góc:24 ↔ nhôm định hình 20x20_600_có lỗ:1
- Mate:72: ke góc:13 ↔ nhôm định hình 20x20_600_có lỗ:1
- Mate:73: nhôm định hình 20x20_700:3 ↔ nhôm định hình 20x20_600_có lỗ:1
- Mate:74: ke góc:12 ↔ nhôm định hình 20x20_600_có lỗ:1
- Mate:75: ke góc:19 ↔ nhôm định hình 20x20_600_có lỗ:1
- Mate:76: ke góc:22 ↔ nhôm định hình 20x20_600_có lỗ:2
- Mate:77: nhôm định hình 20x20_600_có lỗ:2 ↔ nhôm định hình 20x20_700_co lỗ1:1
- Mate:78: nhôm định hình 20x20_600_có lỗ:1 ↔ nhôm định hình 20x20_700_co lỗ1:1
- Flush:74: nhôm định hình 20x20_600_có lỗ:1 ↔ nhôm định hình 20x20_700_co lỗ1:1
- Mate:79: nhôm định hình 20x20_600_có lỗ:1 ↔ nhôm định hình 20x20_700_co lỗ2:1
- Flush:75: nhôm định hình 20x20_600_có lỗ:2 ↔ nhôm định hình 20x20_700_co lỗ2:1
- Mate:80: nhôm định hình 20x20_600_có lỗ:2 ↔ nhôm định hình 20x20_700_co lỗ2:1
- Mate:81: nhôm định hình 20x20_700_co lỗ1:1 ↔ đế trên:1
- Flush:76: nhôm định hình 20x20_700_co lỗ2:1 ↔ đế trên:1
- Mate:82: nhôm định hình 20x20_700_co lỗ2:1 ↔ đế trên:1
- Mate:83: đế trên:1 ↔ nhôm định hình đôi_gá link1:1
- Mate:84: đế trên:1 ↔ nhôm định hình đôi_gá link1:1
- Mate:85: đế trên:1 ↔ nhôm định hình đôi_gá link1:1
- Mate:86: nhôm định hình đôi_gá link1:1 ↔ Hộp trượt vòng bi:1
- Flush:77: nhôm định hình đôi_gá link1:1 ↔ Hộp trượt vòng bi:1
- Mate:88: Hộp trượt vòng bi:1 ↔ trục đai:1
- Mate:89: Hộp trượt vòng bi:1 ↔ trục đai:1
- Mate:90: trục đai:1 ↔ mặt bích:1
- Mate:92: mặt bích:1 ↔ Link1:1
- Mate:93: mặt bích:1 ↔ Link1:1
- Mate:94: mặt bích:1 ↔ Link1:1
- Mate:95: đế trên:1 ↔ nhôm định hình đôi_gá link1:3
- Mate:96: đế trên:1 ↔ nhôm định hình đôi_gá link1:3
- Mate:97: đế trên:1 ↔ nhôm định hình đôi_gá link1:3
- Mate:98: đế trên:1 ↔ nhôm định hình đôi_gá link1:2
- Mate:99: đế trên:1 ↔ nhôm định hình đôi_gá link1:2
- Mate:100: đế trên:1 ↔ nhôm định hình đôi_gá link1:2
- Mate:101: nhôm định hình đôi_gá link1:2 ↔ Hộp trượt vòng bi:2
- Flush:78: nhôm định hình đôi_gá link1:2 ↔ Hộp trượt vòng bi:2
- Mate:103: nhôm định hình đôi_gá link1:3 ↔ Hộp trượt vòng bi:3
- Flush:79: nhôm định hình đôi_gá link1:3 ↔ Hộp trượt vòng bi:3
- Mate:105: Hộp trượt vòng bi:3 ↔ trục đai:2
- Mate:106: Hộp trượt vòng bi:3 ↔ trục đai:2
- Mate:107: Hộp trượt vòng bi:2 ↔ trục đai:3
- Mate:109: trục đai:3 ↔ mặt bích:3
- Mate:111: trục đai:2 ↔ mặt bích:2
- Mate:113: mặt bích:3 ↔ Link1:2
- Mate:114: mặt bích:3 ↔ Link1:2
- Mate:115: mặt bích:3 ↔ Link1:2
- Mate:116: mặt bích:2 ↔ Link1:3
- Mate:117: mặt bích:2 ↔ Link1:3
- Mate:118: mặt bích:2 ↔ Link1:3
- Mate:119: trục đai:2 ↔ khóa trục:1
- Mate:120: Hộp trượt vòng bi:3 ↔ khóa trục:1
- Mate:121: trục đai:1 ↔ khóa trục:2
- Mate:122: Hộp trượt vòng bi:1 ↔ khóa trục:2
- Mate:123: trục đai:3 ↔ khóa trục:3
- Mate:124: Hộp trượt vòng bi:2 ↔ khóa trục:3
- Mate:125: Link1:3 ↔ chốt khớp nối:1
- Mate:126: Link1:3 ↔ chốt khớp nối:1
- Mate:127: Link1:3 ↔ chốt khớp nối:3
- Mate:128: Link1:3 ↔ chốt khớp nối:3
- Mate:129: Link1:1 ↔ chốt khớp nối:6
- Mate:130: Link1:1 ↔ chốt khớp nối:6
- Mate:131: Link1:1 ↔ chốt khớp nối:2
- Mate:132: Link1:1 ↔ chốt khớp nối:2
- Mate:133: Link1:2 ↔ chốt khớp nối:5
- Mate:134: Link1:2 ↔ chốt khớp nối:5
- Mate:135: Link1:2 ↔ chốt khớp nối:4
- Mate:136: Link1:2 ↔ chốt khớp nối:4
- Mate:208: trục đai:2 ↔ mặt bích:2
- Mate:209: trục đai:1 ↔ mặt bích:1
- Mate:210: chốt khớp nối:6 ↔ linh2_mawts traau:1
- Mate:211: chốt khớp nối:6 ↔ linh2_mawts traau:1
- Mate:212: chốt khớp nối:2 ↔ linh2_mawts traau:6
- Mate:213: chốt khớp nối:2 ↔ linh2_mawts traau:6
- Mate:214: chốt khớp nối:3 ↔ linh2_mawts traau:5
- Mate:215: chốt khớp nối:1 ↔ linh2_mawts traau:5
- Mate:216: chốt khớp nối:3 ↔ linh2_mawts traau:3
- Mate:217: chốt khớp nối:3 ↔ linh2_mawts traau:3
- Mate:218: chốt khớp nối:4 ↔ linh2_mawts traau:2
- Mate:219: chốt khớp nối:4 ↔ linh2_mawts traau:2
- Mate:220: chốt khớp nối:5 ↔ linh2_mawts traau:4
- Mate:221: chốt khớp nối:5 ↔ linh2_mawts traau:4
- Mate:222: linh2_mawts traau:5 ↔ Base_E_buffer:1
- Mate:223: linh2_mawts traau:5 ↔ Base_E_buffer:1
- Mate:224: linh2_mawts traau:3 ↔ Base_E_buffer:1
- Mate:225: linh2_mawts traau:4 ↔ Base_E_buffer:1
- Mate:226: linh2_mawts traau:4 ↔ Base_E_buffer:1
- Mate:227: linh2_mawts traau:2 ↔ Base_E_buffer:1
- Mate:228: linh2_mawts traau:2 ↔ Base_E_buffer:1
- Mate:229: linh2_mawts traau:4 ↔ Base_E_buffer:1
- Mate:230: linh2_mawts traau:5 ↔ Base_E_buffer:1
- Mate:231: linh2_mawts traau:3 ↔ Base_E_buffer:1
- Mate:232: linh2_mawts traau:1 ↔ Base_E_buffer:1
- Mate:233: linh2_mawts traau:1 ↔ Base_E_buffer:1
- Mate:234: linh2_mawts traau:6 ↔ Base_E_buffer:1
- Mate:235: linh2_mawts traau:6 ↔ Base_E_buffer:1
- Flush:80: nhôm định hình đôi_gá link1:2 ↔ Hộp trượt vòng bi:2
- Flush:81: nhôm định hình đôi_gá link1:3 ↔ Hộp trượt vòng bi:3
- Flush:82: nhôm định hình đôi_gá link1:1 ↔ Hộp trượt vòng bi:1
- Mate:236: nhôm định hình đôi_gá link1:1 ↔ đế gá step:1
- Flush:83: nhôm định hình đôi_gá link1:1 ↔ đế gá step:1
- Flush:84: nhôm định hình đôi_gá link1:1 ↔ đế gá step:1
- Mate:237: nema23:1 ↔ đế gá step:1
- Mate:239: nhôm định hình đôi_gá link1:3 ↔ đế gá step:2
- Flush:86: nhôm định hình đôi_gá link1:3 ↔ đế gá step:2
- Flush:87: nhôm định hình đôi_gá link1:2 ↔ đế gá step:3
- Mate:242: nhôm định hình đôi_gá link1:2 ↔ đế gá step:3
- Flush:88: nhôm định hình đôi_gá link1:2 ↔ đế gá step:3
- Mate:243: đế gá step:3 ↔ nema23:3
- Flush:94: nhôm định hình đôi_gá link1:3 ↔ đế gá step:2
- Mate:249: đế gá step:2 ↔ nema23:4
- Mate:251: nema23:1 ↔ đế gá step:1
- Flush:95: đế gá step:3 ↔ nema23:3
- Flush:96: đế gá step:2 ↔ nema23:4
- Mate:252: nema23:1 ↔ GT2_20T:2
- Flush:97: nema23:1 ↔ GT2_20T:2
- Mate:253: nema23:4 ↔ GT2_20T:1
- Flush:98: nema23:4 ↔ GT2_20T:1
- Mate:254: nema23:3 ↔ GT2_20T:3
- Flush:99: nema23:3 ↔ GT2_20T:3
- Mate:255: trục đai:3 ↔ GT2_60:2
- Flush:100: GT2_20T:3 ↔ GT2_60:2
- Mate:256: trục đai:1 ↔ GT2_60:3
- Flush:101: GT2_20T:2 ↔ GT2_60:3
- Mate:257: trục đai:2 ↔ GT2_60:1
- Flush:102: GT2_20T:1 ↔ GT2_60:1
- Insert:59: đế gá step:2 ↔ AS 1427 H - Metric M4 x 8:1
- Insert:60: đế gá step:2 ↔ AS 1427 H - Metric M4 x 8:2
- Insert:61: đế gá step:2 ↔ AS 1427 H - Metric M4 x 8:3
- Insert:62: đế gá step:2 ↔ AS 1427 H - Metric M4 x 8:4
- Insert:63: đế gá step:1 ↔ AS 1427 H - Metric M4 x 8:5
- Insert:64: đế gá step:1 ↔ AS 1427 H - Metric M4 x 8:6
- Insert:65: đế gá step:1 ↔ AS 1427 H - Metric M4 x 8:7
- Insert:66: đế gá step:1 ↔ AS 1427 H - Metric M4 x 8:8
- Insert:67: đế gá step:3 ↔ AS 1427 H - Metric M4 x 8:9
- Insert:68: đế gá step:3 ↔ AS 1427 H - Metric M4 x 8:10
- Insert:69: đế gá step:3 ↔ AS 1427 H - Metric M4 x 8:11
- Insert:70: đế gá step:3 ↔ AS 1427 H - Metric M4 x 8:12
- Insert:71: Link1:3 ↔ AS 1427 H - Metric M2.5 x 4:1
- Insert:72: Link1:3 ↔ AS 1427 H - Metric M2.5 x 4:2
- Insert:73: Link1:3 ↔ AS 1427 H - Metric M2.5 x 4:3
- Insert:74: Link1:3 ↔ AS 1427 H - Metric M2.5 x 4:4
- Insert:75: Link1:2 ↔ AS 1427 H - Metric M2.5 x 4:5
- Insert:76: Link1:2 ↔ AS 1427 H - Metric M2.5 x 4:6
- Insert:77: Link1:2 ↔ AS 1427 H - Metric M2.5 x 4:7
- Insert:78: Link1:2 ↔ AS 1427 H - Metric M2.5 x 4:8
- Insert:79: Link1:1 ↔ AS 1427 H - Metric M2.5 x 4:9
- Insert:80: Link1:1 ↔ AS 1427 H - Metric M2.5 x 4:10
- Insert:81: Link1:1 ↔ AS 1427 H - Metric M2.5 x 4:11
- Insert:82: Link1:1 ↔ AS 1427 H - Metric M2.5 x 4:12
- Mate:258: khóa trục:1 ↔ AS 1427 H - Metric M3.5 x 5:1
- Mate:259: khóa trục:2 ↔ AS 1427 H - Metric M3.5 x 5:2
- Mate:260: khóa trục:3 ↔ AS 1427 H - Metric M3.5 x 5:3
- Insert:83: Hộp trượt vòng bi:2 ↔ AS 1427 H - Metric M3 x 5:1
- Insert:84: Hộp trượt vòng bi:2 ↔ AS 1427 H - Metric M3 x 5:2
- Insert:85: Hộp trượt vòng bi:2 ↔ AS 1427 H - Metric M3 x 5:3
- Insert:86: Hộp trượt vòng bi:2 ↔ AS 1427 H - Metric M3 x 5:4
- Mate:261: Hộp trượt vòng bi:3 ↔ AS 1427 H - Metric M3 x 5:5
- Mate:262: Hộp trượt vòng bi:3 ↔ AS 1427 H - Metric M3 x 5:5
- Insert:87: Hộp trượt vòng bi:3 ↔ AS 1427 H - Metric M3 x 5:6
- Insert:88: Hộp trượt vòng bi:3 ↔ AS 1427 H - Metric M3 x 5:7
- Insert:89: Hộp trượt vòng bi:3 ↔ AS 1427 H - Metric M3 x 16:1
- Insert:90: Hộp trượt vòng bi:1 ↔ AS 1427 H - Metric M3 x 16:2
- Insert:91: Hộp trượt vòng bi:1 ↔ AS 1427 H - Metric M3 x 16:3
- Insert:92: Hộp trượt vòng bi:1 ↔ AS 1427 H - Metric M3 x 16:4
- Insert:93: Hộp trượt vòng bi:1 ↔ AS 1427 H - Metric M3 x 16:5
- Insert:94: đế trên:1 ↔ AS 1427 H - Metric M4 x 6:1
- Insert:95: đế trên:1 ↔ AS 1427 H - Metric M4 x 6:2
- Insert:96: đế trên:1 ↔ AS 1427 H - Metric M4 x 6:3
- Insert:97: đế trên:1 ↔ AS 1427 H - Metric M4 x 6:4
- Insert:98: đế trên:1 ↔ AS 1427 H - Metric M4 x 6:5
- Insert:99: đế trên:1 ↔ AS 1427 H - Metric M4 x 6:6
- Insert:100: đế trên:1 ↔ AS 1427 H - Metric M4 x 6:7
- Insert:101: đế trên:1 ↔ AS 1427 H - Metric M4 x 6:8
- Insert:103: đế trên:1 ↔ AS 1427 H - Metric M4 x 6:10
- Insert:104: nhôm định hình 20x20_700_co lỗ2:1 ↔ AS 1427 H - Metric M4 x 6:11
- Insert:105: nhôm định hình 20x20_700_co lỗ2:1 ↔ AS 1427 H - Metric M4 x 6:12
- Insert:106: nhôm định hình 20x20_700_co lỗ2:1 ↔ AS 1427 H - Metric M4 x 6:13
- Insert:107: đế trên:1 ↔ AS 1427 H - Metric M4 x 6:14
- Insert:108: đế trên:1 ↔ AS 1427 H - Metric M4 x 6:15
- Insert:109: đế trên:1 ↔ AS 1427 H - Metric M4 x 6:16
- Insert:110: đế trên:1 ↔ AS 1427 H - Metric M4 x 6:17
- Insert:111: đế trên:1 ↔ AS 1427 H - Metric M4 x 6:18
- Insert:124: linh2_mawts traau:6 ↔ Broached Hexagon Socket Button Head Cap Screw - Metric M3 x 0.5 x 45:1
- Insert:125: linh2_mawts traau:6 ↔ Broached Hexagon Socket Button Head Cap Screw - Metric M3 x 0.5 x 45:2
- Insert:126: linh2_mawts traau:3 ↔ Broached Hexagon Socket Button Head Cap Screw - Metric M3 x 0.5 x 45:3
- Mate:263: linh2_mawts traau:3 ↔ Broached Hexagon Socket Button Head Cap Screw - Metric M3 x 0.5 x 45:4
- Mate:264: linh2_mawts traau:3 ↔ Broached Hexagon Socket Button Head Cap Screw - Metric M3 x 0.5 x 45:4
- Insert:127: linh2_mawts traau:4 ↔ Broached Hexagon Socket Button Head Cap Screw - Metric M3 x 0.5 x 45:5
- Insert:128: linh2_mawts traau:4 ↔ Broached Hexagon Socket Button Head Cap Screw - Metric M3 x 0.5 x 45:6
- Insert:129: linh2_mawts traau:2 ↔ ANSI B18.2.4.2M M3.5x0.6:1
- Insert:130: linh2_mawts traau:5 ↔ ANSI B18.2.4.2M M3.5x0.6:2
- Insert:131: linh2_mawts traau:1 ↔ ANSI B18.2.4.2M M3.5x0.6:3
- Insert:132: linh2_mawts traau:1 ↔ ANSI B18.2.4.2M M3.5x0.6:4
- Insert:133: linh2_mawts traau:2 ↔ ANSI B18.2.4.2M M3.5x0.6:5
- Insert:134: linh2_mawts traau:5 ↔ ANSI B18.2.4.2M M3.5x0.6:6
- Flush:103: nhôm định hình đôi_gá link1:1 ↔ Part1:3
- Flush:104: nhôm định hình đôi_gá link1:1 ↔ Part1:3
- Mate:265: nhôm định hình đôi_gá link1:1 ↔ Part1:3
- Mate:266: nhôm định hình đôi_gá link1:2 ↔ Part1:1
- Flush:105: nhôm định hình đôi_gá link1:2 ↔ Part1:1
- Flush:106: nhôm định hình đôi_gá link1:2 ↔ Part1:1
- Mate:267: nhôm định hình đôi_gá link1:3 ↔ Part1:2
- Flush:107: nhôm định hình đôi_gá link1:3 ↔ Part1:2
- Flush:108: nhôm định hình đôi_gá link1:3 ↔ Part1:2
- Insert:135: Part1:2 ↔ AS 1427 H - Metric M4 x 10:1
- Insert:136: Part1:2 ↔ AS 1427 H - Metric M4 x 10:2
- Insert:137: Part1:3 ↔ AS 1427 H - Metric M4 x 10:3
- Insert:138: Part1:3 ↔ AS 1427 H - Metric M4 x 10:4
- Insert:139: Part1:1 ↔ AS 1427 H - Metric M4 x 10:5
- Insert:140: Part1:1 ↔ AS 1427 H - Metric M4 x 10:6
- Mate:268: Part1:3 ↔ công tắc hành trình:3
- Mate:269: Part1:3 ↔ công tắc hành trình:3
- Mate:270: Part1:3 ↔ công tắc hành trình:3
- Mate:271: Part1:2 ↔ công tắc hành trình:1
- Mate:272: Part1:2 ↔ công tắc hành trình:1
- Mate:273: Part1:2 ↔ công tắc hành trình:1
- Mate:274: Part1:1 ↔ công tắc hành trình:2
- Mate:275: Part1:1 ↔ công tắc hành trình:2
- Mate:276: Part1:1 ↔ công tắc hành trình:2
- Insert:141: đế trên:1 ↔ AS 1427 H - Metric M4 x 16:1
- Insert:142: đế trên:1 ↔ AS 1427 H - Metric M4 x 16:2
- Insert:143: đế trên:1 ↔ AS 1427 H - Metric M4 x 16:3
- Insert:144: đế trên:1 ↔ AS 1427 H - Metric M4 x 16:4
- Insert:145: đế trên:1 ↔ AS 1427 H - Metric M4 x 16:5
- Insert:146: đế trên:1 ↔ AS 1427 H - Metric M4 x 16:6
- Insert:147: đế trên:1 ↔ AS 1427 H - Metric M4 x 16:7
- Insert:148: đế trên:1 ↔ AS 1427 H - Metric M4 x 16:8
- Insert:149: đế trên:1 ↔ AS 1427 H - Metric M4 x 16:9
- Insert:150: đế trên:1 ↔ AS 1427 H - Metric M4 x 16:10
- Insert:151: đế trên:1 ↔ AS 1427 H - Metric M4 x 16:11
- Insert:152: đế trên:1 ↔ AS 1427 H - Metric M4 x 10:7
- Insert:153: đế trên:1 ↔ AS 1427 H - Metric M4 x 16:12
- Insert:154: công tắc hành trình:1 ↔ AS 1427 H - Metric M3 x 5:8
- Insert:155: công tắc hành trình:1 ↔ AS 1427 H - Metric M3 x 5:9
- Insert:156: công tắc hành trình:2 ↔ AS 1427 H - Metric M3 x 5:10
- Insert:157: công tắc hành trình:2 ↔ AS 1427 H - Metric M3 x 5:11
- Insert:158: công tắc hành trình:3 ↔ AS 1427 H - Metric M3 x 5:12
- Insert:159: công tắc hành trình:3 ↔ AS 1427 H - Metric M3 x 5:13
